# Autodesk Inventor assembly: Ring Gear
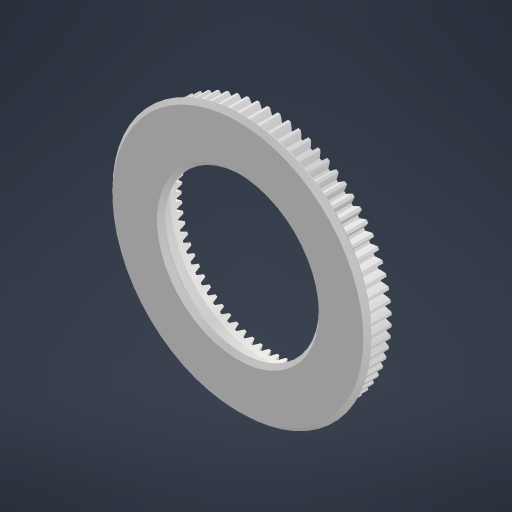
[picture p0: Inventor's stored thumbnail of the model, 512x512]
Saved by Autodesk Inventor 2024 (Build 280153000, 153)
## iProperties
Created: 2023-08-14
Part Number: Ring Gear
Document SubType Name: Assembly
Designer: Izack Waczko
Author: Izack Waczko
## Documents named in this file (4)
- C:\Users\izack\Robotics\CAD\Custom-Modules-CAD\Differential Swerve Drive V1\Differential Swerve Drive Parts\Ring Gear.iam
- C:\Users\izack\Robotics\CAD\Custom-Modules-CAD\Differential Swerve Drive V1\Ring Gear Base.ipt
- C:\Users\izack\Robotics\CAD\Custom-Modules-CAD\Differential Swerve Drive V1\Differential Swerve Drive V1\Design Accelerator\Bevel Gear11.ipt
- C:\Users\izack\Robotics\CAD\Custom-Modules-CAD\Differential Swerve Drive V1\Differential Swerve Drive Parts\Bottom_Ring.ipt
## Components (3 placed, 3 different names)
1. Ring Gear Base:1 — Mate:1, Mate:2, Rigid:1, Flush:1
2. Bevel Gear1:1 — Mate:1, Mate:2, Rigid:1
3. Bottom_Ring:1 — Flush:1
## Relationships (4: Mate 2, WeldJoint 1, Flush 1)
- Mate:1: Ring Gear Base:1 ↔ Bevel Gear1:1
- Mate:2: Ring Gear Base:1 ↔ Bevel Gear1:1
- Rigid:1 [WeldJoint]: Ring Gear Base:1 ↔ Bevel Gear1:1
- Flush:1: Ring Gear Base:1 ↔ Bottom_Ring:1
